# Autodesk Inventor assembly: Load_Cell_Total
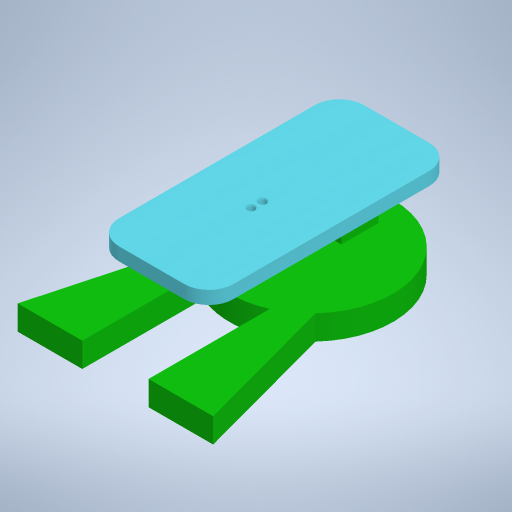
[picture p0: Inventor's stored thumbnail of the model, 512x512]
Saved by Autodesk Inventor 2023 (Build 270158000, 158)
## iProperties
Created: 2023-03-13
Part Number: Load_Cell_Total
Document SubType Name: Assembly
Designer: Inteli
Author: Inteli
## Documents named in this file (4)
- C:\Users\Inteli\Documents\GitHub\grupo1\src\3d_models\Celula_De_Carga\Load_Cell_Total.iam
- C:\Users\Inteli\Documents\GitHub\grupo1\src\3d_models\Celula_De_Carga\Base inferior(suporte).ipt
- C:\Users\Inteli\Documents\GitHub\grupo1\src\3d_models\Celula_De_Carga\Base superior(suporte).ipt
- C:\Users\Inteli\Documents\GitHub\grupo1\src\3d_models\Celula_De_Carga\celula de carga.ipt
## Components (3 placed, 3 different names)
1. Base inferior(suporte):1 — Insert:1, Insert:2
2. Base superior(suporte):1 — Mate:1
3. celula de carga:1 — Mate:1, Insert:1, Insert:2
## Relationships (3: Insert 2, Mate 1)
- Mate:1: Base superior(suporte):1 ↔ celula de carga:1
- Insert:1: Base inferior(suporte):1 ↔ celula de carga:1
- Insert:2: Base inferior(suporte):1 ↔ celula de carga:1
